# Autodesk Inventor assembly: jezek_v_kleci
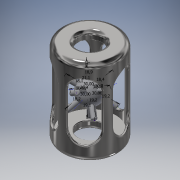
[picture p0: Inventor's stored thumbnail of the model, 180x180]
Saved by Autodesk Inventor 2018 (Build 220112000, 112)
## iProperties
Created: 2024-01-23
Part Number: jezek_v_kleci
Material: Všeobecné
Document SubType Name: Assembly
Designer: 42073
Author: 42073
## Documents named in this file (3)
- C:\Users\42073\Documents\2_Škola\inventor\F1\jezek_v_kleci.iam
- C:\Users\42073\Documents\2_Škola\inventor\F1\klec.ipt
- C:\Users\42073\Documents\2_Škola\inventor\F1\jezek v.ipt
## Components (2 placed, 2 different names)
1. klec:1 — Proti sobě:1, Stejný směr:1
2. jezek v:1 — Proti sobě:1, Stejný směr:1
## Relationships (2: Mate 1, Flush 1)
- Proti sobě:1 [Mate]: klec:1 ↔ jezek v:1
- Stejný směr:1 [Flush] (16.621 mm): klec:1 ↔ jezek v:1
